# Autodesk Inventor assembly: GearLiftProto
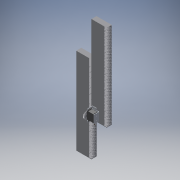
[picture p0: Inventor's stored thumbnail of the model, 180x180]
Saved by Autodesk Inventor 2017 (Build 210142000, 142)
## iProperties
Created: 2017-11-15
Part Number: GearLiftProto
Document SubType Name: Assembly
Designer: User
Author: User
## Documents named in this file (5)
- C:\Robotics\CAD\2017-18_CAD\Prototypes\GearLiftProto.iam
- C:\Robotics\CAD\2017-18_CAD\Prototypes\GearLiftProtoPart1.ipt
- C:\Robotics\CAD\COTSParts\Tetrix\Tetrix servo 180.ipt
- C:\Robotics\CAD\COTSParts\Tetrix\Tetrix Gear 40T.ipt
- C:\Robotics\CAD\COTSParts\Tetrix\39060_txm-standard servo bracket.ipt
## Components (5 placed, 4 different names)
1. GearLiftProtoPart1:1 — Mate:1, Flush:1, Mate:3
2. GearLiftProtoPart1:2 — Mate:1, Flush:1, Mate:14, Flush:2
3. Tetrix servo 180:2 — Mate:7, Mate:8, Mate:9, Mate:10, Mate:12, Mate:13
4. Tetrix Gear 40T:1 — Mate:3, Mate:10, Mate:12, Mate:13
5. 39060_txm-standard servo bracket:2 — Mate:7, Mate:8, Mate:9, Mate:14, Flush:2
## Relationships (11: Mate 9, Flush 2)
- Mate:1: GearLiftProtoPart1:1 ↔ GearLiftProtoPart1:2
- Flush:1: GearLiftProtoPart1:1 ↔ GearLiftProtoPart1:2
- Mate:3 (2.54 mm): GearLiftProtoPart1:1 ↔ Tetrix Gear 40T:1
- Mate:7: Tetrix servo 180:2 ↔ 39060_txm-standard servo bracket:2
- Mate:8: Tetrix servo 180:2 ↔ 39060_txm-standard servo bracket:2
- Mate:9: Tetrix servo 180:2 ↔ 39060_txm-standard servo bracket:2
- Mate:10: Tetrix servo 180:2 ↔ Tetrix Gear 40T:1
- Mate:12: Tetrix servo 180:2 ↔ Tetrix Gear 40T:1
- Mate:13: Tetrix servo 180:2 ↔ Tetrix Gear 40T:1
- Mate:14: GearLiftProtoPart1:2 ↔ 39060_txm-standard servo bracket:2
- Flush:2: GearLiftProtoPart1:2 ↔ 39060_txm-standard servo bracket:2
